# Autodesk Inventor assembly: FrontWheelBrakeAssembly
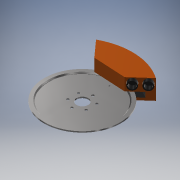
[picture p0: Inventor's stored thumbnail of the model, 180x180]
Saved by Autodesk Inventor 2019.4 (Build 234330000, 330)
## iProperties
Created: 2020-10-08
Part Number: FrontWheelBrakeAssembly
Document SubType Name: Assembly
Designer: Federico
Author: Federico
## Documents named in this file (3)
- C:\Users\Federico\Desktop\236\Project\CARMODEL\FrontWheelBrakeAssembly.iam
- C:\Users\Federico\Desktop\236\Project\CARMODEL\DiskForBrakes.ipt
- C:\Users\Federico\Desktop\236\Project\CARMODEL\Calliper.ipt
## Components (2 placed, 2 different names)
1. DiskForBrakes:1 — Rotational:1
2. Calliper:1 — Rotational:1
## Relationships (1: RevoluteJoint 1)
- Rotational:1 [RevoluteJoint]: DiskForBrakes:1 ↔ Calliper:1
